# Autodesk Inventor assembly: Leg
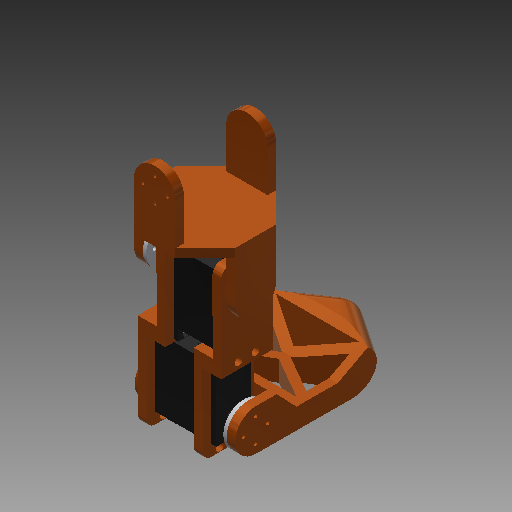
[picture p0: Inventor's stored thumbnail of the model, 512x512]
Saved by Autodesk Inventor 2017 (Build 210142000, 142)
## iProperties
Created: 2017-01-26
Part Number: Leg
Document SubType Name: Assembly
Designer: Alexander Miller
Author: Alexander Miller
## Documents named in this file (4)
- D:\Daten\Documents\Git\Hexapod\3DParts\HexPi_v2\Leg.iam
- D:\Daten\Documents\Git\Hexapod\3DParts\HexPi_v2\Hip.iam
- D:\Daten\Documents\Git\Hexapod\3DParts\HexPi_v2\Thigh.iam
- D:\Daten\Documents\Git\Hexapod\3DParts\HexPi_v2\Tibia.ipt
## Components (3 placed, 3 different names)
1. Hip:1 [sub-assembly] — Rigid:1
2. Thigh:1 [sub-assembly] — Rigid:1, Rigid:2
3. Tibia:1 — Rigid:2
## Relationships (2: WeldJoint 2)
- Rigid:1 [WeldJoint]: Hip:1 ↔ Thigh:1
- Rigid:2 [WeldJoint]: Thigh:1 ↔ Tibia:1
